# Autodesk Inventor assembly: tip
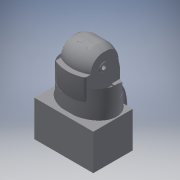
[picture p0: Inventor's stored thumbnail of the model, 180x180]
Saved by Autodesk Inventor 2019 (Build 230136000, 136)
## iProperties
Created: 2024-08-26
Part Number: tip
Material: Generisch
Document SubType Name: Assembly
Designer: nic
Author: nic
## Documents named in this file (3)
- C:\Users\Nicolas Frick\Sync\OneDrive\wtm\nicol_rh8d\inventor\tip.iam
- C:\Users\Nicolas Frick\Sync\OneDrive\wtm\nicol_rh8d\inventor\tip.ipt
- C:\Users\Nicolas Frick\Sync\OneDrive\wtm\nicol_rh8d\inventor\tip_plate.ipt
## Components (2 placed, 2 different names)
1. tip:1 — Passend:1, Passend:2, Fluchtend:1
2. tip_plate:1 — Fluchtend:2
## Relationships (4: Mate 2, Flush 2)
- Passend:1 [Mate]: tip:1
- Passend:2 [Mate]: tip:1
- Fluchtend:1 [Flush]: tip:1
- Fluchtend:2 [Flush]: tip_plate:1
